# Autodesk Inventor assembly: Dynamixel MX-106
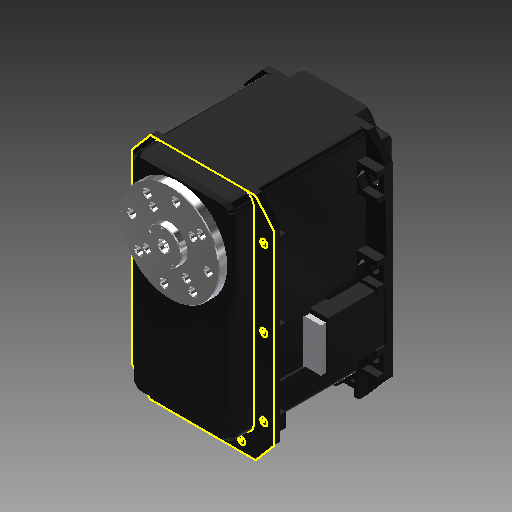
[picture p0: Inventor's stored thumbnail of the model, 512x512]
Saved by Autodesk Inventor 2019 (Build 230136000, 136)
## iProperties
Created: 2020-03-18
Part Number: Dynamixel MX-106
Material: Типовые
Document SubType Name: Assembly
Designer: Петров Иван
Author: Петров Иван
## Documents named in this file (3)
- E:\IVAN\Ivan_desktop\Kvantorium\Competitions\INOP_2020\hardware\SCARA(Dynamixels)\components\Dynamixel MX-106.iam
- E:\IVAN\Ivan_desktop\Kvantorium\Competitions\INOP_2020\hardware\SCARA(Dynamixels)\components\Сервомотор Dynamixel MX-106R.ipt
- E:\IVAN\Ivan_desktop\Kvantorium\Competitions\INOP_2020\hardware\SCARA(Dynamixels)\components\Колесо сервомотора.ipt
## Components (2 placed, 2 different names)
1. Сервомотор Dynamixel MX-106R:1 — Совмещение:1, Совмещение:2
2. Колесо сервомотора:1 — Совмещение:1, Совмещение:2
## Relationships (2: Mate 2)
- Совмещение:1 [Mate]: Сервомотор Dynamixel MX-106R:1 ↔ Колесо сервомотора:1
- Совмещение:2 [Mate]: Сервомотор Dynamixel MX-106R:1 ↔ Колесо сервомотора:1
